# Autodesk Inventor assembly: Почти готово_CPY
(part 2 of 3)
592. Винт ГОСТ 11738-84 M 10x35:3
593. Шайба  ГОСТ 11371-78 13:6
594. Винт ГОСТ 11738-84 M 10x35:4
595. Шайба  ГОСТ 11371-78 13:7
596. Винт ГОСТ 11738-84 M 10x35:5
597. Шайба  ГОСТ 11371-78 13:8
598. Винт ГОСТ 11738-84 M 10x35:6
599. Шайба  ГОСТ 11371-78 13:9
600. Винт ГОСТ 11738-84 M 10x35:7
601. Шайба  ГОСТ 11371-78 13:10
602. Винт ГОСТ 11738-84 M 10x35:8
603. Шайба  ГОСТ 11371-78 13:11
604. Винт ГОСТ 11738-84 M 10x30:1 — Жесткий:131
605. Шайба  ГОСТ 11371-78 13:2 — Жесткий:130, Жесткий:131
606. Винт ГОСТ 11738-84 M 10x30:2
607. Шайба  ГОСТ 11371-78 13:12
608. Винт ГОСТ 11738-84 M 10x30:3
609. Шайба  ГОСТ 11371-78 13:13
610. Винт ГОСТ 11738-84 M 10x30:4
611. Шайба  ГОСТ 11371-78 13:14
612. Винт ГОСТ 11738-84 M 10x30:5
613. Шайба  ГОСТ 11371-78 13:15
614. Винт ГОСТ 11738-84 M 10x30:6
615. Шайба  ГОСТ 11371-78 13:16
616. Винт ГОСТ 11738-84 M 10x30:7
617. Шайба  ГОСТ 11371-78 13:17
618. Винт ГОСТ 11738-84 M 10x30:8
619. Шайба  ГОСТ 11371-78 13:18
620. Шайба  ГОСТ 11371-78 13:4 — Жесткий:134, Жесткий:135
621. Винт ГОСТ 11738-84 M 10x25:2 — Жесткий:135
622. Шайба  ГОСТ 11371-78 13:19
623. Винт ГОСТ 11738-84 M 10x25:3
624. Шайба  ГОСТ 11371-78 13:20
625. Винт ГОСТ 11738-84 M 10x25:4
626. Шайба  ГОСТ 11371-78 13:21
627. Винт ГОСТ 11738-84 M 10x25:5
628. Шайба  ГОСТ 11371-78 13:22
629. Винт ГОСТ 11738-84 M 10x25:6
630. Шайба  ГОСТ 11371-78 13:23
631. Винт ГОСТ 11738-84 M 10x25:7
632. Шайба  ГОСТ 11371-78 13:24
633. Винт ГОСТ 11738-84 M 10x25:8
634. Шайба  ГОСТ 11371-78 13:25
635. Винт ГОСТ 11738-84 M 10x25:9
636. Винт ГОСТ 11738-84 M 10x25:1 — Жесткий:133
637. Шайба  ГОСТ 11371-78 13:3 — Жесткий:133, Жесткий:132
638. Винт ГОСТ 11738-84 M 10x25:10
639. Шайба  ГОСТ 11371-78 13:26
640. Винт ГОСТ 11738-84 M 10x25:11
641. Шайба  ГОСТ 11371-78 13:27
642. Винт ГОСТ 11738-84 M 10x25:12
643. Шайба  ГОСТ 11371-78 13:28
644. Винт ГОСТ 11738-84 M 10x25:13
645. Шайба  ГОСТ 11371-78 13:29
646. Винт ГОСТ 11738-84 M 10x25:14
647. Шайба  ГОСТ 11371-78 13:30
648. Винт ГОСТ 11738-84 M 10x25:15
649. Шайба  ГОСТ 11371-78 13:31
650. Винт ГОСТ 11738-84 M 10x25:16
651. Шайба  ГОСТ 11371-78 13:32
652. Шпилька ГОСТ 22034-76 M20-6g×50:2 — Жесткий:122, Жесткий:124, Жесткий:123
653. Гайка ГОСТ 15521-70 M20:2 — Жесткий:124
654. Шайба ГОСТ 10450-78 19:2 — Жесткий:123
655. Шпилька ГОСТ 22034-76 M20-6g×50:14
656. Гайка ГОСТ 15521-70 M20:14
657. Шайба ГОСТ 10450-78 19:14
658. Шпилька ГОСТ 22034-76 M20-6g×50:15
659. Гайка ГОСТ 15521-70 M20:15
660. Шайба ГОСТ 10450-78 19:15
661. Шпилька ГОСТ 22034-76 M20-6g×50:16
662. Гайка ГОСТ 15521-70 M20:16
663. Шайба ГОСТ 10450-78 19:16
664. Шпилька ГОСТ 22034-76 M20-6g×50:17
665. Гайка ГОСТ 15521-70 M20:17
666. Шайба ГОСТ 10450-78 19:17
667. Шпилька ГОСТ 22034-76 M20-6g×50:18
668. Гайка ГОСТ 15521-70 M20:18
669. Шайба ГОСТ 10450-78 19:18
670. Шпилька ГОСТ 22034-76 M20-6g×50:19
671. Гайка ГОСТ 15521-70 M20:19
672. Шайба ГОСТ 10450-78 19:19
673. Шпилька ГОСТ 22034-76 M20-6g×50:20
674. Гайка ГОСТ 15521-70 M20:20
675. Шайба ГОСТ 10450-78 19:20
676. Шпилька ГОСТ 22034-76 M20-6g×50:21
677. Гайка ГОСТ 15521-70 M20:21
678. Шайба ГОСТ 10450-78 19:21
679. Шпилька ГОСТ 22034-76 M20-6g×50:22
680. Гайка ГОСТ 15521-70 M20:22
681. Шайба ГОСТ 10450-78 19:22
682. Гайка ГОСТ 15521-70 M20:3 — Жесткий:198
683. Шпилька ГОСТ 22034-76 M20-6g×50:3 — Жесткий:198, Жесткий:199
684. Шайба ГОСТ 10450-78 19:3 — Жесткий:199
685. Гайка ГОСТ 15521-70 M20:23
686. Шпилька ГОСТ 22034-76 M20-6g×50:23
687. Шайба ГОСТ 10450-78 19:23
688. Гайка ГОСТ 15521-70 M20:24
689. Шпилька ГОСТ 22034-76 M20-6g×50:24
690. Шайба ГОСТ 10450-78 19:24
691. Гайка ГОСТ 15521-70 M20:25
692. Шпилька ГОСТ 22034-76 M20-6g×50:25
693. Шайба ГОСТ 10450-78 19:25
694. Гайка ГОСТ 15521-70 M20:26
695. Шпилька ГОСТ 22034-76 M20-6g×50:26
696. Шайба ГОСТ 10450-78 19:26
697. Гайка ГОСТ 15521-70 M20:27
698. Шпилька ГОСТ 22034-76 M20-6g×50:27
699. Шайба ГОСТ 10450-78 19:27
700. Гайка ГОСТ 15521-70 M20:28
701. Шпилька ГОСТ 22034-76 M20-6g×50:28
702. Шайба ГОСТ 10450-78 19:28
703. Гайка ГОСТ 15521-70 M20:29
704. Шпилька ГОСТ 22034-76 M20-6g×50:29
705. Шайба ГОСТ 10450-78 19:29
706. Гайка ГОСТ 15521-70 M20:30
707. Шпилька ГОСТ 22034-76 M20-6g×50:30
708. Шайба ГОСТ 10450-78 19:30
709. Гайка ГОСТ 15521-70 M20:31
710. Шпилька ГОСТ 22034-76 M20-6g×50:31
711. Шайба ГОСТ 10450-78 19:31
712. Шпилька ГОСТ 22034-76 M20-6g×50:4 — Жесткий:200, Жесткий:201
713. Гайка ГОСТ 15521-70 M20:4 — Жесткий:200
714. Шайба ГОСТ 10450-78 19:4 — Жесткий:201
715. Шпилька ГОСТ 22034-76 M20-6g×50:32
716. Гайка ГОСТ 15521-70 M20:32
717. Шайба ГОСТ 10450-78 19:32
718. Шпилька ГОСТ 22034-76 M20-6g×50:33
719. Гайка ГОСТ 15521-70 M20:33
720. Шайба ГОСТ 10450-78 19:33
721. Шпилька ГОСТ 22034-76 M20-6g×50:34
722. Гайка ГОСТ 15521-70 M20:34
723. Шайба ГОСТ 10450-78 19:34
724. Шпилька ГОСТ 22034-76 M20-6g×50:35
725. Гайка ГОСТ 15521-70 M20:35
726. Шайба ГОСТ 10450-78 19:35
727. Шпилька ГОСТ 22034-76 M20-6g×50:36
728. Гайка ГОСТ 15521-70 M20:36
729. Шайба ГОСТ 10450-78 19:36
730. Шпилька ГОСТ 22034-76 M20-6g×50:37
731. Гайка ГОСТ 15521-70 M20:37
732. Шайба ГОСТ 10450-78 19:37
733. Шпилька ГОСТ 22034-76 M20-6g×50:38
734. Гайка ГОСТ 15521-70 M20:38
735. Шайба ГОСТ 10450-78 19:38
736. Шпилька ГОСТ 22034-76 M20-6g×50:39
737. Гайка ГОСТ 15521-70 M20:39
738. Шайба ГОСТ 10450-78 19:39
739. Шпилька ГОСТ 22034-76 M20-6g×50:40
740. Гайка ГОСТ 15521-70 M20:40
741. Шайба ГОСТ 10450-78 19:40
## Component patterns: (16 elements, first: Шпилька ГОСТ 22038-76 M20-6g×85:1 + Шайба ГОСТ 10450-78 21:1 + Гайка ГОСТ 15524-70 M20:1), (10 elements, first: Гайка ГОСТ 15521-70 M20:1 + Шпилька ГОСТ 22034-76 M20-6g×50:1 + Шайба ГОСТ 10450-78 19:1), (16 elements, first: Шпилька ГОСТ 22038-76 M24-6g×70:1 + Гайка ГОСТ 15524-70 M24:1 + Шайба  ГОСТ 11371-78 25:1), (8 elements, first: Винт ГОСТ 11738-84 M 10x35:1 + Шайба  ГОСТ 11371-78 13:1), (8 elements, first: Винт ГОСТ 11738-84 M 10x30:1 + Шайба  ГОСТ 11371-78 13:2), (8 elements, first: Шайба  ГОСТ 11371-78 13:4 + Винт ГОСТ 11738-84 M 10x25:2), (8 elements, first: Винт ГОСТ 11738-84 M 10x25:1 + Шайба  ГОСТ 11371-78 13:3), (10 elements, first: Шпилька ГОСТ 22034-76 M20-6g×50:2 + Гайка ГОСТ 15521-70 M20:2 + Шайба ГОСТ 10450-78 19:2), (10 elements, first: Гайка ГОСТ 15521-70 M20:3 + Шпилька ГОСТ 22034-76 M20-6g×50:3 + Шайба ГОСТ 10450-78 19:3), (10 elements, first: Шпилька ГОСТ 22034-76 M20-6g×50:4 + Гайка ГОСТ 15521-70 M20:4 + Шайба ГОСТ 10450-78 19:4)
## Relationships (407: WeldJoint 394, Flush 7, Mate 2, CylindricalJoint 2, RevoluteJoint 2)
- Совмещение:1 [Mate] (115 mm): Верхняя часть поршня_CPY:1 ↔ Крышка цилиндра 1_CPY:1
- Заподлицо:1 [Flush] (449.5 mm): Шайба  ГОСТ 11371-78 25:1
- Совмещение:2 [Mate] (449.5 mm): Шайба  ГОСТ 11371-78 25:2
- Заподлицо:2 [Flush] (-412.5 mm): Цилиндр2_CPY:1
- Заподлицо:3 [Flush] (-307 mm): Деталь6_CPY:1
- Заподлицо:5 [Flush]: Фонарь_CPY:1 ↔ Прокладка крышки фонаря 1_CPY:1
- Заподлицо:4 [Flush]: Фонарь_CPY:1 ↔ Прокладка крышки фонаря 1_CPY:1
- Заподлицо:7 [Flush]: Фонарь_CPY:1 ↔ Прокладка крышки фонаря 2_CPY:1
- Заподлицо:6 [Flush]: Фонарь_CPY:1 ↔ Прокладка крышки фонаря 2_CPY:1
- Цилиндрический:2 [CylindricalJoint]: Фонарь_CPY:1 ↔ Башмак_CPY:1
- Жесткий:4 [WeldJoint]: Башмак_CPY:1 ↔ Крейцкопф_CPY:1
- Жесткий:1 [WeldJoint]: Втулка под палец_CPY:1 ↔ Крейцкопф_CPY:1
- Жесткий:3 [WeldJoint]: Втулка палец шатун_CPY:1 ↔ Втулка под палец_CPY:2
- Жесткий:2 [WeldJoint]: Крейцкопф_CPY:1 ↔ Втулка под палец_CPY:2
- Жесткий:5 [WeldJoint]: Крейцкопф_CPY:1 ↔ Башмак_CPY:2
- С поворотом:1 [RevoluteJoint]: Втулка под палец_CPY:1 ↔ Палец_CPY:1
- Жесткий:7 [WeldJoint]: Палец_CPY:1 ↔ Стопорное кольцо_CPY:1
- Жесткий:6 [WeldJoint]: Палец_CPY:1 ↔ Стопорное кольцо_CPY:2
- Жесткий:14 [WeldJoint]: Гайка шток-поршень_CPY:1 ↔ Кольцо поршень-шток верх_CPY:1
- Жесткий:13 [WeldJoint]: Верхняя часть поршня_CPY:1 ↔ Кольцо поршень-шток верх_CPY:1
- Жесткий:9 [WeldJoint]: Верхняя часть поршня_CPY:1 ↔ Кольцо поршня_CPY:1
- С поворотом:3 [RevoluteJoint]: Корпус дросселя_CPY:1 ↔ Корпус сальника_CPY:1
- Жесткий:16 [WeldJoint]: Втулка_CPY:1 ↔ Крышка цилиндра 1_CPY:1
- Жесткий:70 [WeldJoint] (-2 mm): Фонарь_CPY:1 ↔ Крышка цилиндра 2_CPY:1
- Жесткий:12 [WeldJoint]: Кольцо поршень-шток низ_CPY:1 ↔ Нижняя часть поршня_CPY:1
- Жесткий:8 [WeldJoint]: Верхняя часть поршня_CPY:1 ↔ Нижняя часть поршня_CPY:1
- Жесткий:21 [WeldJoint]: Нижняя часть поршня_CPY:1 ↔ Опорное кольцо_CPY:1
- Жесткий:27 [WeldJoint]: Кольцо сальника_CPY:1 ↔ Пружина сальника_CPY:1
- Жесткий:79 [WeldJoint]: Крышка цилиндра 2_CPY:1 ↔ Цилиндр2_CPY:1
- Жесткий:23 [WeldJoint] (1 mm): Крышка стакана_CPY:1 ↔ Цилиндр2_CPY:1
- Жесткий:15 [WeldJoint]: Втулка_CPY:1 ↔ Цилиндр2_CPY:1
- Жесткий:11 [WeldJoint]: Нижняя часть поршня_CPY:1 ↔ Кольцо поршня_CPY:2
- Цилиндрический:1 [CylindricalJoint]: Втулка_CPY:1 ↔ Кольцо поршня_CPY:3
- Жесткий:10 [WeldJoint]: Нижняя часть поршня_CPY:1 ↔ Кольцо поршня_CPY:3
- Жесткий:80 [WeldJoint] (-2 mm): Цилиндр2_CPY:1 ↔ Клапан1_CPY:1
- Жесткий:18 [WeldJoint]: Цилиндр2_CPY:1 ↔ Прокладка клапана_CPY:1
- Жесткий:81 [WeldJoint] (-22 mm): Цилиндр2_CPY:1 ↔ Стакан1_CPY:1
- Жесткий:20 [WeldJoint]: Верхняя часть поршня_CPY:1 ↔ Опорное кольцо_CPY:2
- Жесткий:26 [WeldJoint]: Корпус дросселя_CPY:1 ↔ Дроссельное кольцо_CPY:1
- Жесткий:25 [WeldJoint] (2 mm): Пружина дросселя_CPY:1 ↔ Дроссельное кольцо_CPY:1
- Жесткий:32 [WeldJoint]: Корпус сальника_CPY:1 ↔ Кольцо сальника_CPY:2
- Жесткий:31 [WeldJoint]: Кольцо сальника_CPY:1 ↔ Кольцо сальника_CPY:2
- Жесткий:28 [WeldJoint]: Кольцо сальника_CPY:2 ↔ Пружина сальника_CPY:2
- Жесткий:30 [WeldJoint]: Кольцо сальника_CPY:1 ↔ Кольцо сальника_CPY:3
- Жесткий:29 [WeldJoint]: Кольцо сальника_CPY:3 ↔ Пружина сальника_CPY:3
- Жесткий:57 [WeldJoint]: Корпус сальника_CPY:1 ↔ Корпус сальника_CPY:2
- Жесткий:33 [WeldJoint]: Кольцо сальника_CPY:4 ↔ Пружина сальника_CPY:4
- Жесткий:38 [WeldJoint]: Корпус сальника_CPY:2 ↔ Кольцо сальника_CPY:5
- Жесткий:37 [WeldJoint]: Кольцо сальника_CPY:4 ↔ Кольцо сальника_CPY:5
- Жесткий:34 [WeldJoint]: Кольцо сальника_CPY:5 ↔ Пружина сальника_CPY:5
- Жесткий:36 [WeldJoint]: Кольцо сальника_CPY:4 ↔ Кольцо сальника_CPY:6
- Жесткий:35 [WeldJoint]: Кольцо сальника_CPY:6 ↔ Пружина сальника_CPY:6
- Жесткий:58 [WeldJoint]: Корпус сальника_CPY:2 ↔ Корпус сальника_CPY:3
- Жесткий:39 [WeldJoint]: Кольцо сальника_CPY:7 ↔ Пружина сальника_CPY:7
- Жесткий:44 [WeldJoint]: Корпус сальника_CPY:3 ↔ Кольцо сальника_CPY:8
- Жесткий:43 [WeldJoint]: Кольцо сальника_CPY:7 ↔ Кольцо сальника_CPY:8
- Жесткий:40 [WeldJoint]: Кольцо сальника_CPY:8 ↔ Пружина сальника_CPY:8
- Жесткий:42 [WeldJoint]: Кольцо сальника_CPY:7 ↔ Кольцо сальника_CPY:9
- Жесткий:41 [WeldJoint]: Кольцо сальника_CPY:9 ↔ Пружина сальника_CPY:9
- Жесткий:59 [WeldJoint]: Корпус сальника_CPY:3 ↔ Корпус сальника_CPY:4
- Жесткий:45 [WeldJoint]: Кольцо сальника_CPY:10 ↔ Пружина сальника_CPY:10
- Жесткий:50 [WeldJoint]: Корпус сальника_CPY:4 ↔ Кольцо сальника_CPY:11
- Жесткий:49 [WeldJoint]: Кольцо сальника_CPY:10 ↔ Кольцо сальника_CPY:11
- Жесткий:46 [WeldJoint]: Кольцо сальника_CPY:11 ↔ Пружина сальника_CPY:11
- Жесткий:48 [WeldJoint]: Кольцо сальника_CPY:10 ↔ Кольцо сальника_CPY:12
- Жесткий:47 [WeldJoint]: Кольцо сальника_CPY:12 ↔ Пружина сальника_CPY:12
- Жесткий:60 [WeldJoint]: Корпус сальника_CPY:4 ↔ Корпус сальника_CPY:5
- Жесткий:51 [WeldJoint]: Кольцо сальника_CPY:13 ↔ Пружина сальника_CPY:13
- Жесткий:56 [WeldJoint]: Корпус сальника_CPY:5 ↔ Кольцо сальника_CPY:14
- Жесткий:55 [WeldJoint]: Кольцо сальника_CPY:13 ↔ Кольцо сальника_CPY:14
- Жесткий:52 [WeldJoint]: Кольцо сальника_CPY:14 ↔ Пружина сальника_CPY:14
- Жесткий:54 [WeldJoint]: Кольцо сальника_CPY:13 ↔ Кольцо сальника_CPY:15
- Жесткий:53 [WeldJoint]: Кольцо сальника_CPY:15 ↔ Пружина сальника_CPY:15
- Жесткий:62 [WeldJoint] (-1 mm): Корпус дросселя_CPY:1 ↔ Уплотнительное кольцо_CPY:1
- Жесткий:61 [WeldJoint] (1 mm): Крышка цилиндра 2_CPY:1 ↔ Уплотнительное кольцо_CPY:1
- Жесткий:63 [WeldJoint]: Кольцо сальника_CPY:16 ↔ Пружина сальника_CPY:16
- Жесткий:67 [WeldJoint]: Кольцо сальника_CPY:16 ↔ Кольцо сальника_CPY:17
- Жесткий:64 [WeldJoint]: Кольцо сальника_CPY:17 ↔ Пружина сальника_CPY:17
- Жесткий:66 [WeldJoint]: Кольцо сальника_CPY:16 ↔ Кольцо сальника_CPY:18
- Жесткий:65 [WeldJoint]: Кольцо сальника_CPY:18 ↔ Пружина сальника_CPY:18
- Жесткий:69 [WeldJoint]: Фонарь_CPY:1 ↔ Уплотнение фонарь_CPY:1
- Жесткий:77 [WeldJoint]: Корпус сальника_CPY:5 ↔ Корпус сальника_CPY:6
- Жесткий:71 [WeldJoint]: Кольцо сальника_CPY:19 ↔ Пружина сальника_CPY:19
- Жесткий:76 [WeldJoint]: Корпус сальника_CPY:6 ↔ Кольцо сальника_CPY:20
- Жесткий:75 [WeldJoint]: Кольцо сальника_CPY:19 ↔ Кольцо сальника_CPY:20
- Жесткий:72 [WeldJoint]: Кольцо сальника_CPY:20 ↔ Пружина сальника_CPY:20
- Жесткий:74 [WeldJoint]: Кольцо сальника_CPY:19 ↔ Кольцо сальника_CPY:21
- Жесткий:73 [WeldJoint]: Кольцо сальника_CPY:21 ↔ Пружина сальника_CPY:21
- Жесткий:78 [WeldJoint] (3 mm): Крышка цилиндра 2_CPY:1 ↔ Крышка сальников_CPY:1
- Жесткий:95 [WeldJoint]: Корпус сальника перегородка 1_CPY:1 ↔ Крышка перегородки11_CPY:1
- Жесткий:94 [WeldJoint]: Фонарь_CPY:1 ↔ Крышка перегородки11_CPY:1
- Жесткий:96 [WeldJoint]: Корпус сальника перегородка 1_CPY:1 ↔ Крышка перегородки12_CPY:1
- Жесткий:104 [WeldJoint]: Корпус маслосъемника_CPY:1 ↔ Крышка перегородки21_CPY:1
- Жесткий:103 [WeldJoint]: Кольцо сальника_CPY:17 ↔ Крышка перегородки21_CPY:1
- Жесткий:98 [WeldJoint]: Фонарь_CPY:1 ↔ Крышка перегородки21_CPY:1
- Жесткий:105 [WeldJoint]: Крышка перегородки21_CPY:1 ↔ Крышка перегородки22_CPY:1
- Жесткий:99 [WeldJoint] (-1 mm): Маслосъемная пружина_CPY:1 ↔ Маслосъемное кольцо_CPY:1
- Жесткий:97 [WeldJoint]: Фонарь_CPY:1 ↔ Придав перегородки1_CPY:1
- Жесткий:82 [WeldJoint]: Кольцо сальника_CPY:22 ↔ Пружина сальника_CPY:22
- Жесткий:87 [WeldJoint]: Корпус сальника перегородка 1_CPY:1 ↔ Кольцо сальника_CPY:23
- Жесткий:86 [WeldJoint]: Кольцо сальника_CPY:22 ↔ Кольцо сальника_CPY:23
- Жесткий:83 [WeldJoint]: Кольцо сальника_CPY:23 ↔ Пружина сальника_CPY:23
- Жесткий:85 [WeldJoint]: Кольцо сальника_CPY:22 ↔ Кольцо сальника_CPY:24
- Жесткий:84 [WeldJoint]: Кольцо сальника_CPY:24 ↔ Пружина сальника_CPY:24
- Жесткий:88 [WeldJoint]: Кольцо сальника_CPY:25 ↔ Пружина сальника_CPY:25
- Жесткий:93 [WeldJoint]: Корпус сальника перегородка 1_CPY:1 ↔ Кольцо сальника_CPY:26
- Жесткий:92 [WeldJoint]: Кольцо сальника_CPY:25 ↔ Кольцо сальника_CPY:26
- Жесткий:89 [WeldJoint]: Кольцо сальника_CPY:26 ↔ Пружина сальника_CPY:26
- Жесткий:91 [WeldJoint]: Кольцо сальника_CPY:25 ↔ Кольцо сальника_CPY:27
- Жесткий:90 [WeldJoint]: Кольцо сальника_CPY:27 ↔ Пружина сальника_CPY:27
- Жесткий:102 [WeldJoint]: Корпус маслосъемника_CPY:1 ↔ Маслосъемное кольцо_CPY:2
- Жесткий:101 [WeldJoint]: Маслосъемное кольцо_CPY:1 ↔ Маслосъемное кольцо_CPY:2
- Жесткий:100 [WeldJoint] (-1 mm): Маслосъемная пружина_CPY:2 ↔ Маслосъемное кольцо_CPY:2
- Жесткий:106 [WeldJoint]: Фонарь_CPY:1 ↔ Придав перегородки1_CPY:2
- Жесткий:110 [WeldJoint] (-3.5 mm): Гайка шток_CPY:1 ↔ Шток_CPY:1
- Жесткий:107 [WeldJoint] (4.75 mm): Гайка шток-поршень_CPY:1 ↔ Шток_CPY:1
- Жесткий:207 [WeldJoint]: Фланецгайка_CPY:1 ↔ Прокладка крейцкопф_CPY:1
- Жесткий:206 [WeldJoint]: Крейцкопф_CPY:1 ↔ Прокладка крейцкопф_CPY:1
- Жесткий:112 [WeldJoint]: Крышка цилиндра 1_CPY:1 ↔ Шайба  ГОСТ 11371-78 25:1
- Жесткий:113 [WeldJoint] (-8.75 mm): Шпилька ГОСТ 22038-76 M24-6g×70:1 ↔ Гайка ГОСТ 15524-70 M24:1
- Жесткий:111 [WeldJoint]: Цилиндр2_CPY:1 ↔ Шпилька ГОСТ 22038-76 M24-6g×70:1
- Жесткий:114 [WeldJoint] (-8.75 mm): Шпилька ГОСТ 22038-76 M24-6g×70:2 ↔ Гайка ГОСТ 15524-70 M24:2
- Жесткий:116 [WeldJoint] (-2 mm): Цилиндр2_CPY:1 ↔ Клапан1_CPY:2
- Жесткий:115 [WeldJoint]: Цилиндр2_CPY:1 ↔ Прокладка клапана_CPY:2
- Жесткий:117 [WeldJoint] (-22 mm): Цилиндр2_CPY:1 ↔ Стакан1_CPY:2
- Жесткий:118 [WeldJoint] (1 mm): Цилиндр2_CPY:1 ↔ Крышка стакана_CPY:2
- Жесткий:119 [WeldJoint] (-1 mm): Цилиндр2_CPY:1 ↔ Шпилька ГОСТ 22034-76 M20-6g×50:1
- Жесткий:121 [WeldJoint] (-2.5 mm): Гайка ГОСТ 15521-70 M20:1 ↔ Шпилька ГОСТ 22034-76 M20-6g×50:1
- Жесткий:120 [WeldJoint] (-20 mm): Шпилька ГОСТ 22034-76 M20-6g×50:1 ↔ Шайба ГОСТ 10450-78 19:1
- Жесткий:122 [WeldJoint]: Цилиндр2_CPY:1 ↔ Шпилька ГОСТ 22034-76 M20-6g×50:2
- Жесткий:124 [WeldJoint] (-2.25 mm): Шпилька ГОСТ 22034-76 M20-6g×50:2 ↔ Гайка ГОСТ 15521-70 M20:2
- Жесткий:123 [WeldJoint] (-20 mm): Шпилька ГОСТ 22034-76 M20-6g×50:2 ↔ Шайба ГОСТ 10450-78 19:2
- Жесткий:127 [WeldJoint] (-2 mm): Фонарь_CPY:1 ↔ Гайка ГОСТ 15524-70 M20:1
- Жесткий:126 [WeldJoint] (-32 mm): Шпилька ГОСТ 22038-76 M20-6g×85:1 ↔ Шайба ГОСТ 10450-78 21:1
- Жесткий:125 [WeldJoint]: Крышка цилиндра 2_CPY:1 ↔ Шпилька ГОСТ 22038-76 M20-6g×85:1
- Жесткий:130 [WeldJoint]: Крышка перегородки22_CPY:1 ↔ Шайба  ГОСТ 11371-78 13:2
- Жесткий:134 [WeldJoint]: Придав перегородки1_CPY:1 ↔ Шайба  ГОСТ 11371-78 13:4
- Жесткий:128 [WeldJoint]: Крышка перегородки12_CPY:1 ↔ Шайба  ГОСТ 11371-78 13:1
- Жесткий:135 [WeldJoint]: Шайба  ГОСТ 11371-78 13:4 ↔ Винт ГОСТ 11738-84 M 10x25:2
- Жесткий:133 [WeldJoint]: Винт ГОСТ 11738-84 M 10x25:1 ↔ Шайба  ГОСТ 11371-78 13:3
- Жесткий:132 [WeldJoint]: Придав перегородки1_CPY:2 ↔ Шайба  ГОСТ 11371-78 13:3
- Жесткий:129 [WeldJoint]: Винт ГОСТ 11738-84 M 10x35:1 ↔ Шайба  ГОСТ 11371-78 13:1
- Жесткий:131 [WeldJoint]: Винт ГОСТ 11738-84 M 10x30:1 ↔ Шайба  ГОСТ 11371-78 13:2
- Жесткий:138 [WeldJoint] (-38 mm): Шпилька ГОСТ 22038-76 M24-6g×80:1 ↔ Гайка ГОСТ 15524-70 M24:18
- Жесткий:137 [WeldJoint] (-38 mm): Шпилька ГОСТ 22038-76 M24-6g×80:1 ↔ Шайба  ГОСТ 11371-78 28:1
- Жесткий:140 [WeldJoint] (-38 mm): Шпилька ГОСТ 22038-76 M24-6g×80:2 ↔ Гайка ГОСТ 15524-70 M24:19
- Жесткий:163 [WeldJoint]: Фонарь_CPY:1 ↔ Шайба  ГОСТ 11371-78 28:2
- Жесткий:139 [WeldJoint] (-38 mm): Шпилька ГОСТ 22038-76 M24-6g×80:2 ↔ Шайба  ГОСТ 11371-78 28:2
- Жесткий:142 [WeldJoint] (-38 mm): Шпилька ГОСТ 22038-76 M24-6g×80:3 ↔ Гайка ГОСТ 15524-70 M24:20
- Жесткий:165 [WeldJoint]: Фонарь_CPY:1 ↔ Шайба  ГОСТ 11371-78 28:3
- Жесткий:141 [WeldJoint] (-38 mm): Шпилька ГОСТ 22038-76 M24-6g×80:3 ↔ Шайба  ГОСТ 11371-78 28:3
- Жесткий:144 [WeldJoint] (-38 mm): Шпилька ГОСТ 22038-76 M24-6g×80:4 ↔ Гайка ГОСТ 15524-70 M24:21
- Жесткий:166 [WeldJoint]: Фонарь_CPY:1 ↔ Шайба  ГОСТ 11371-78 28:4
- Жесткий:143 [WeldJoint] (-38 mm): Шпилька ГОСТ 22038-76 M24-6g×80:4 ↔ Шайба  ГОСТ 11371-78 28:4
- Жесткий:146 [WeldJoint] (-38 mm): Шпилька ГОСТ 22038-76 M24-6g×80:5 ↔ Гайка ГОСТ 15524-70 M24:22
- Жесткий:164 [WeldJoint]: Фонарь_CPY:1 ↔ Шайба  ГОСТ 11371-78 28:5
- Жесткий:145 [WeldJoint] (-38 mm): Шпилька ГОСТ 22038-76 M24-6g×80:5 ↔ Шайба  ГОСТ 11371-78 28:5
- Жесткий:148 [WeldJoint] (-38 mm): Шпилька ГОСТ 22038-76 M24-6g×80:6 ↔ Гайка ГОСТ 15524-70 M24:23
- Жесткий:171 [WeldJoint]: Фонарь_CPY:1 ↔ Шайба  ГОСТ 11371-78 28:6
- Жесткий:147 [WeldJoint] (-38 mm): Шпилька ГОСТ 22038-76 M24-6g×80:6 ↔ Шайба  ГОСТ 11371-78 28:6
- Жесткий:150 [WeldJoint] (-38 mm): Шпилька ГОСТ 22038-76 M24-6g×80:7 ↔ Гайка ГОСТ 15524-70 M24:24
- Жесткий:173 [WeldJoint]: Фонарь_CPY:1 ↔ Шайба  ГОСТ 11371-78 28:7
- Жесткий:149 [WeldJoint] (-38 mm): Шпилька ГОСТ 22038-76 M24-6g×80:7 ↔ Шайба  ГОСТ 11371-78 28:7
- Жесткий:152 [WeldJoint] (-38 mm): Шпилька ГОСТ 22038-76 M24-6g×80:8 ↔ Гайка ГОСТ 15524-70 M24:25
- Жесткий:174 [WeldJoint]: Фонарь_CPY:1 ↔ Шайба  ГОСТ 11371-78 28:8
- Жесткий:151 [WeldJoint] (-38 mm): Шпилька ГОСТ 22038-76 M24-6g×80:8 ↔ Шайба  ГОСТ 11371-78 28:8
- Жесткий:154 [WeldJoint] (-38 mm): Шпилька ГОСТ 22038-76 M24-6g×80:9 ↔ Гайка ГОСТ 15524-70 M24:26
- Жесткий:172 [WeldJoint]: Фонарь_CPY:1 ↔ Шайба  ГОСТ 11371-78 28:9
- Жесткий:153 [WeldJoint] (-38 mm): Шпилька ГОСТ 22038-76 M24-6g×80:9 ↔ Шайба  ГОСТ 11371-78 28:9
- Жесткий:156 [WeldJoint] (-38 mm): Шпилька ГОСТ 22038-76 M24-6g×80:10 ↔ Гайка ГОСТ 15524-70 M24:27
- Жесткий:169 [WeldJoint]: Фонарь_CPY:1 ↔ Шайба  ГОСТ 11371-78 28:10
- Жесткий:155 [WeldJoint] (-38 mm): Шпилька ГОСТ 22038-76 M24-6g×80:10 ↔ Шайба  ГОСТ 11371-78 28:10
- Жесткий:158 [WeldJoint] (-38 mm): Шпилька ГОСТ 22038-76 M24-6g×80:11 ↔ Гайка ГОСТ 15524-70 M24:28
- Жесткий:167 [WeldJoint]: Фонарь_CPY:1 ↔ Шайба  ГОСТ 11371-78 28:11
- Жесткий:157 [WeldJoint] (-38 mm): Шпилька ГОСТ 22038-76 M24-6g×80:11 ↔ Шайба  ГОСТ 11371-78 28:11
- Жесткий:160 [WeldJoint] (-38 mm): Шпилька ГОСТ 22038-76 M24-6g×80:12 ↔ Гайка ГОСТ 15524-70 M24:29
- Жесткий:170 [WeldJoint]: Фонарь_CPY:1 ↔ Шайба  ГОСТ 11371-78 28:12
- Жесткий:159 [WeldJoint] (-38 mm): Шпилька ГОСТ 22038-76 M24-6g×80:12 ↔ Шайба  ГОСТ 11371-78 28:12
- Жесткий:162 [WeldJoint] (-38 mm): Шпилька ГОСТ 22038-76 M24-6g×80:13 ↔ Гайка ГОСТ 15524-70 M24:30
- Жесткий:168 [WeldJoint]: Фонарь_CPY:1 ↔ Шайба  ГОСТ 11371-78 28:13
- Жесткий:161 [WeldJoint] (-38 mm): Шпилька ГОСТ 22038-76 M24-6g×80:13 ↔ Шайба  ГОСТ 11371-78 28:13
- Жесткий:176 [WeldJoint] (-38 mm): Шпилька ГОСТ 22038-76 M24-6g×80:14 ↔ Гайка ГОСТ 15524-70 M24:31
- Жесткий:192 [WeldJoint]: Фонарь_CPY:1 ↔ Шайба  ГОСТ 11371-78 28:14
- Жесткий:175 [WeldJoint] (-38 mm): Шпилька ГОСТ 22038-76 M24-6g×80:14 ↔ Шайба  ГОСТ 11371-78 28:14
- Жесткий:178 [WeldJoint] (-38 mm): Шпилька ГОСТ 22038-76 M24-6g×80:15 ↔ Гайка ГОСТ 15524-70 M24:32
- Жесткий:197 [WeldJoint]: Фонарь_CPY:1 ↔ Шайба  ГОСТ 11371-78 28:15
- Жесткий:177 [WeldJoint] (-38 mm): Шпилька ГОСТ 22038-76 M24-6g×80:15 ↔ Шайба  ГОСТ 11371-78 28:15
- Жесткий:180 [WeldJoint] (-38 mm): Шпилька ГОСТ 22038-76 M24-6g×80:16 ↔ Гайка ГОСТ 15524-70 M24:33
- Жесткий:191 [WeldJoint]: Фонарь_CPY:1 ↔ Шайба  ГОСТ 11371-78 28:16
- Жесткий:179 [WeldJoint] (-38 mm): Шпилька ГОСТ 22038-76 M24-6g×80:16 ↔ Шайба  ГОСТ 11371-78 28:16
- Жесткий:184 [WeldJoint] (-38 mm): Шпилька ГОСТ 22038-76 M24-6g×80:17 ↔ Гайка ГОСТ 15524-70 M24:34
- Жесткий:196 [WeldJoint]: Фонарь_CPY:1 ↔ Шайба  ГОСТ 11371-78 28:17
- Жесткий:183 [WeldJoint] (-38 mm): Шпилька ГОСТ 22038-76 M24-6g×80:17 ↔ Шайба  ГОСТ 11371-78 28:17
- Жесткий:186 [WeldJoint] (-38 mm): Шпилька ГОСТ 22038-76 M24-6g×80:18 ↔ Гайка ГОСТ 15524-70 M24:35
- Жесткий:194 [WeldJoint]: Фонарь_CPY:1 ↔ Шайба  ГОСТ 11371-78 28:18
- Жесткий:185 [WeldJoint] (-38 mm): Шпилька ГОСТ 22038-76 M24-6g×80:18 ↔ Шайба  ГОСТ 11371-78 28:18
- Жесткий:188 [WeldJoint] (-38 mm): Шпилька ГОСТ 22038-76 M24-6g×80:19 ↔ Гайка ГОСТ 15524-70 M24:36
- Жесткий:193 [WeldJoint]: Фонарь_CPY:1 ↔ Шайба  ГОСТ 11371-78 28:19
- Жесткий:187 [WeldJoint] (-38 mm): Шпилька ГОСТ 22038-76 M24-6g×80:19 ↔ Шайба  ГОСТ 11371-78 28:19
- Жесткий:190 [WeldJoint] (-38 mm): Шпилька ГОСТ 22038-76 M24-6g×80:20 ↔ Гайка ГОСТ 15524-70 M24:37
- Жесткий:195 [WeldJoint]: Фонарь_CPY:1 ↔ Шайба  ГОСТ 11371-78 28:20
- Жесткий:189 [WeldJoint] (-38 mm): Шпилька ГОСТ 22038-76 M24-6g×80:20 ↔ Шайба  ГОСТ 11371-78 28:20
- Жесткий:198 [WeldJoint] (-2.5 mm): Гайка ГОСТ 15521-70 M20:3 ↔ Шпилька ГОСТ 22034-76 M20-6g×50:3
- Жесткий:199 [WeldJoint] (-20 mm): Шпилька ГОСТ 22034-76 M20-6g×50:3 ↔ Шайба ГОСТ 10450-78 19:3
- Жесткий:200 [WeldJoint] (-2.25 mm): Шпилька ГОСТ 22034-76 M20-6g×50:4 ↔ Гайка ГОСТ 15521-70 M20:4
- Жесткий:201 [WeldJoint] (-20 mm): Шпилька ГОСТ 22034-76 M20-6g×50:4 ↔ Шайба ГОСТ 10450-78 19:4
- Жесткий:202 [WeldJoint]: Цилиндр2_CPY:1 ↔ Деталь5_CPY:1
- Жесткий:203 [WeldJoint]: Деталь5_CPY:1 ↔ Деталь6_CPY:1
- Жесткий:204 [WeldJoint]: Цилиндр2_CPY:1 ↔ Деталь5_CPY:2
- Жесткий:205 [WeldJoint]: Деталь5_CPY:2 ↔ Деталь6_CPY:2
- Жесткий:208 [WeldJoint]: Крейцкопф_CPY:1 ↔ Шпилька ГОСТ 22038-76 M20-6g×85:2
- Жесткий:209 [WeldJoint]: Крейцкопф_CPY:1 ↔ Шпилька ГОСТ 22038-76 M20-6g×85:3
- Жесткий:211 [WeldJoint] (-26 mm): Шпилька ГОСТ 22038-76 M20-6g×85:2 ↔ Гайка ГОСТ 15524-70 M20:2
- Жесткий:210 [WeldJoint] (-26 mm): Шпилька ГОСТ 22038-76 M20-6g×85:2 ↔ Шайба  ГОСТ 11371-78 23:1
- Жесткий:213 [WeldJoint] (-2 mm): Шпилька ГОСТ 22038-76 M20-6g×85:3 ↔ Гайка ГОСТ 15524-70 M20:3
- Жесткий:212 [WeldJoint] (-26 mm): Шпилька ГОСТ 22038-76 M20-6g×85:3 ↔ Шайба  ГОСТ 11371-78 23:2
- Жесткий:239 [WeldJoint]: Деталь6_CPY:1 ↔ Болт ГОСТ Р 50274-92 M8-6g×16-F:1
- Жесткий:233 [WeldJoint]: Деталь6_CPY:1 ↔ Болт ГОСТ Р 50274-92 M8-6g×16-F:2
- Жесткий:232 [WeldJoint]: Деталь6_CPY:1 ↔ Болт ГОСТ Р 50274-92 M8-6g×16-F:3
- Жесткий:214 [WeldJoint]: Деталь6_CPY:1 ↔ Болт ГОСТ Р 50274-92 M8-6g×16-F:4
- Жесткий:215 [WeldJoint]: Деталь6_CPY:1 ↔ Болт ГОСТ Р 50274-92 M8-6g×16-F:5
- Жесткий:223 [WeldJoint]: Деталь6_CPY:1 ↔ Болт ГОСТ Р 50274-92 M8-6g×16-F:6
- Жесткий:222 [WeldJoint]: Деталь6_CPY:1 ↔ Болт ГОСТ Р 50274-92 M8-6g×16-F:7
- Жесткий:240 [WeldJoint]: Деталь6_CPY:1 ↔ Болт ГОСТ Р 50274-92 M8-6g×16-F:8
- Жесткий:238 [WeldJoint]: Деталь6_CPY:1 ↔ Болт ГОСТ Р 50274-92 M8-6g×16-F:9
- Жесткий:236 [WeldJoint]: Деталь6_CPY:1 ↔ Болт ГОСТ Р 50274-92 M8-6g×16-F:10
- Жесткий:218 [WeldJoint]: Деталь6_CPY:1 ↔ Болт ГОСТ Р 50274-92 M8-6g×16-F:11
- Жесткий:217 [WeldJoint]: Деталь6_CPY:1 ↔ Болт ГОСТ Р 50274-92 M8-6g×16-F:12
- Жесткий:216 [WeldJoint]: Деталь6_CPY:1 ↔ Болт ГОСТ Р 50274-92 M8-6g×16-F:13
- Жесткий:237 [WeldJoint]: Деталь6_CPY:1 ↔ Болт ГОСТ Р 50274-92 M8-6g×16-F:14
- Жесткий:235 [WeldJoint]: Деталь6_CPY:1 ↔ Болт ГОСТ Р 50274-92 M8-6g×16-F:15
- Жесткий:234 [WeldJoint]: Деталь6_CPY:1 ↔ Болт ГОСТ Р 50274-92 M8-6g×16-F:16
- Жесткий:227 [WeldJoint]: Деталь6_CPY:1 ↔ Болт ГОСТ Р 50274-92 M8-6g×16-F:17
- Жесткий:226 [WeldJoint]: Деталь6_CPY:1 ↔ Болт ГОСТ Р 50274-92 M8-6g×16-F:18
- Жесткий:225 [WeldJoint]: Деталь6_CPY:1 ↔ Болт ГОСТ Р 50274-92 M8-6g×16-F:19
- Жесткий:241 [WeldJoint]: Деталь6_CPY:1 ↔ Болт ГОСТ Р 50274-92 M8-6g×16-F:20
- Жесткий:244 [WeldJoint]: Деталь6_CPY:1 ↔ Болт ГОСТ Р 50274-92 M8-6g×16-F:21
- Жесткий:231 [WeldJoint]: Деталь6_CPY:1 ↔ Болт ГОСТ Р 50274-92 M8-6g×16-F:22
- Жесткий:229 [WeldJoint]: Деталь6_CPY:1 ↔ Болт ГОСТ Р 50274-92 M8-6g×16-F:23
- Жесткий:228 [WeldJoint]: Деталь6_CPY:1 ↔ Болт ГОСТ Р 50274-92 M8-6g×16-F:24
- Жесткий:224 [WeldJoint]: Деталь6_CPY:1 ↔ Болт ГОСТ Р 50274-92 M8-6g×16-F:25
- Жесткий:243 [WeldJoint]: Деталь6_CPY:1 ↔ Болт ГОСТ Р 50274-92 M8-6g×16-F:26
- Жесткий:242 [WeldJoint]: Деталь6_CPY:1 ↔ Болт ГОСТ Р 50274-92 M8-6g×16-F:27
- Жесткий:219 [WeldJoint]: Деталь6_CPY:1 ↔ Болт ГОСТ Р 50274-92 M8-6g×16-F:28
- Жесткий:221 [WeldJoint]: Деталь6_CPY:1 ↔ Болт ГОСТ Р 50274-92 M8-6g×16-F:29
- Жесткий:220 [WeldJoint]: Деталь6_CPY:1 ↔ Болт ГОСТ Р 50274-92 M8-6g×16-F:30
- Жесткий:245 [WeldJoint]: Деталь6_CPY:1 ↔ Болт ГОСТ Р 50274-92 M8-6g×16-F:31
- Жесткий:230 [WeldJoint]: Деталь6_CPY:1 ↔ Болт ГОСТ Р 50274-92 M8-6g×16-F:32
- Жесткий:246 [WeldJoint]: Крышка фонаря 1_CPY:1 ↔ Прокладка крышки фонаря 1_CPY:1
- Жесткий:247 [WeldJoint]: Крышка фонаря 2_CPY:1 ↔ Прокладка крышки фонаря 2_CPY:1
- Жесткий:249 [WeldJoint]: Крышка фонаря 1_CPY:1 ↔ Болт ГОСТ Р 50274-92 M8-6g×16-F:65
- Жесткий:248 [WeldJoint]: Крышка фонаря 1_CPY:1 ↔ Болт ГОСТ Р 50274-92 M8-6g×16-F:66
- Жесткий:250 [WeldJoint]: Крышка фонаря 1_CPY:1 ↔ Болт ГОСТ Р 50274-92 M8-6g×16-F:67
- Жесткий:251 [WeldJoint]: Крышка фонаря 1_CPY:1 ↔ Болт ГОСТ Р 50274-92 M8-6g×16-F:68
- Жесткий:254 [WeldJoint]: Крышка фонаря 1_CPY:1 ↔ Болт ГОСТ Р 50274-92 M8-6g×16-F:69
- Жесткий:252 [WeldJoint]: Крышка фонаря 1_CPY:1 ↔ Болт ГОСТ Р 50274-92 M8-6g×16-F:70
- Жесткий:258 [WeldJoint]: Крышка фонаря 1_CPY:1 ↔ Болт ГОСТ Р 50274-92 M8-6g×16-F:71
- Жесткий:256 [WeldJoint]: Крышка фонаря 1_CPY:1 ↔ Болт ГОСТ Р 50274-92 M8-6g×16-F:72
- Жесткий:255 [WeldJoint]: Крышка фонаря 1_CPY:1 ↔ Болт ГОСТ Р 50274-92 M8-6g×16-F:73
- Жесткий:253 [WeldJoint]: Крышка фонаря 1_CPY:1 ↔ Болт ГОСТ Р 50274-92 M8-6g×16-F:74
- Жесткий:267 [WeldJoint]: Крышка фонаря 1_CPY:1 ↔ Болт ГОСТ Р 50274-92 M8-6g×16-F:75
- Жесткий:266 [WeldJoint]: Крышка фонаря 1_CPY:1 ↔ Болт ГОСТ Р 50274-92 M8-6g×16-F:76
- Жесткий:269 [WeldJoint]: Крышка фонаря 1_CPY:1 ↔ Болт ГОСТ Р 50274-92 M8-6g×16-F:77
- Жесткий:265 [WeldJoint]: Крышка фонаря 1_CPY:1 ↔ Болт ГОСТ Р 50274-92 M8-6g×16-F:78
- Жесткий:273 [WeldJoint]: Крышка фонаря 1_CPY:1 ↔ Болт ГОСТ Р 50274-92 M8-6g×16-F:79
- Жесткий:271 [WeldJoint]: Крышка фонаря 1_CPY:1 ↔ Болт ГОСТ Р 50274-92 M8-6g×16-F:80
- Жесткий:270 [WeldJoint]: Крышка фонаря 1_CPY:1 ↔ Болт ГОСТ Р 50274-92 M8-6g×16-F:81
- Жесткий:268 [WeldJoint]: Крышка фонаря 1_CPY:1 ↔ Болт ГОСТ Р 50274-92 M8-6g×16-F:82
- Жесткий:257 [WeldJoint]: Крышка фонаря 1_CPY:1 ↔ Болт ГОСТ Р 50274-92 M8-6g×16-F:83
- Жесткий:259 [WeldJoint]: Крышка фонаря 1_CPY:1 ↔ Болт ГОСТ Р 50274-92 M8-6g×16-F:84
- Жесткий:261 [WeldJoint]: Крышка фонаря 1_CPY:1 ↔ Болт ГОСТ Р 50274-92 M8-6g×16-F:85
- Жесткий:264 [WeldJoint]: Крышка фонаря 1_CPY:1 ↔ Болт ГОСТ Р 50274-92 M8-6g×16-F:86
- Жесткий:263 [WeldJoint]: Крышка фонаря 1_CPY:1 ↔ Болт ГОСТ Р 50274-92 M8-6g×16-F:87
- Жесткий:262 [WeldJoint]: Крышка фонаря 1_CPY:1 ↔ Болт ГОСТ Р 50274-92 M8-6g×16-F:88
- Жесткий:260 [WeldJoint]: Крышка фонаря 1_CPY:1 ↔ Болт ГОСТ Р 50274-92 M8-6g×16-F:89
- Жесткий:280 [WeldJoint]: Крышка фонаря 2_CPY:1 ↔ Болт ГОСТ Р 50274-92 M8-6g×16-F:90
- Жесткий:281 [WeldJoint]: Крышка фонаря 2_CPY:1 ↔ Болт ГОСТ Р 50274-92 M8-6g×16-F:91
- Жесткий:279 [WeldJoint]: Крышка фонаря 2_CPY:1 ↔ Болт ГОСТ Р 50274-92 M8-6g×16-F:92
- Жесткий:276 [WeldJoint]: Крышка фонаря 2_CPY:1 ↔ Болт ГОСТ Р 50274-92 M8-6g×16-F:93
- Жесткий:295 [WeldJoint]: Крышка фонаря 2_CPY:1 ↔ Болт ГОСТ Р 50274-92 M8-6g×16-F:94
- Жесткий:296 [WeldJoint]: Крышка фонаря 2_CPY:1 ↔ Болт ГОСТ Р 50274-92 M8-6g×16-F:95
- Жесткий:282 [WeldJoint]: Крышка фонаря 2_CPY:1 ↔ Болт ГОСТ Р 50274-92 M8-6g×16-F:96
- Жесткий:278 [WeldJoint]: Крышка фонаря 2_CPY:1 ↔ Болт ГОСТ Р 50274-92 M8-6g×16-F:97
- Жесткий:277 [WeldJoint]: Крышка фонаря 2_CPY:1 ↔ Болт ГОСТ Р 50274-92 M8-6g×16-F:98
- Жесткий:308 [WeldJoint]: Крышка фонаря 2_CPY:1 ↔ Болт ГОСТ Р 50274-92 M8-6g×16-F:99
- Жесткий:274 [WeldJoint]: Крышка фонаря 1_CPY:1 ↔ Болт ГОСТ Р 50274-92 M8-6g×16-F:100
- Жесткий:272 [WeldJoint]: Крышка фонаря 1_CPY:1 ↔ Болт ГОСТ Р 50274-92 M8-6g×16-F:101
- Жесткий:317 [WeldJoint]: Крышка фонаря 2_CPY:1 ↔ Болт ГОСТ Р 50274-92 M8-6g×16-F:102
- Жесткий:318 [WeldJoint]: Крышка фонаря 2_CPY:1 ↔ Болт ГОСТ Р 50274-92 M8-6g×16-F:103
- Жесткий:316 [WeldJoint]: Крышка фонаря 2_CPY:1 ↔ Болт ГОСТ Р 50274-92 M8-6g×16-F:104
- Жесткий:275 [WeldJoint]: Крышка фонаря 1_CPY:1 ↔ Болт ГОСТ Р 50274-92 M8-6g×16-F:105
- Жесткий:310 [WeldJoint]: Крышка фонаря 2_CPY:1 ↔ Болт ГОСТ Р 50274-92 M8-6g×16-F:106
- Жесткий:294 [WeldJoint]: Крышка фонаря 2_CPY:1 ↔ Болт ГОСТ Р 50274-92 M8-6g×16-F:107
- Жесткий:311 [WeldJoint]: Крышка фонаря 2_CPY:1 ↔ Болт ГОСТ Р 50274-92 M8-6g×16-F:108
- Жесткий:307 [WeldJoint]: Крышка фонаря 2_CPY:1 ↔ Болт ГОСТ Р 50274-92 M8-6g×16-F:109
- Жесткий:313 [WeldJoint]: Крышка фонаря 2_CPY:1 ↔ Болт ГОСТ Р 50274-92 M8-6g×16-F:110
- Жесткий:314 [WeldJoint]: Крышка фонаря 2_CPY:1 ↔ Болт ГОСТ Р 50274-92 M8-6g×16-F:111
- Жесткий:315 [WeldJoint]: Крышка фонаря 2_CPY:1 ↔ Болт ГОСТ Р 50274-92 M8-6g×16-F:112
- Жесткий:293 [WeldJoint]: Крышка фонаря 2_CPY:1 ↔ Болт ГОСТ Р 50274-92 M8-6g×16-F:113
- Жесткий:320 [WeldJoint]: Крышка фонаря 2_CPY:1 ↔ Болт ГОСТ Р 50274-92 M8-6g×16-F:114
- Жесткий:300 [WeldJoint]: Крышка фонаря 2_CPY:1 ↔ Болт ГОСТ Р 50274-92 M8-6g×16-F:115
- Жесткий:299 [WeldJoint]: Крышка фонаря 2_CPY:1 ↔ Болт ГОСТ Р 50274-92 M8-6g×16-F:116
- Жесткий:285 [WeldJoint]: Крышка фонаря 2_CPY:1 ↔ Болт ГОСТ Р 50274-92 M8-6g×16-F:117
- Жесткий:301 [WeldJoint]: Крышка фонаря 2_CPY:1 ↔ Болт ГОСТ Р 50274-92 M8-6g×16-F:118
- Жесткий:291 [WeldJoint]: Крышка фонаря 2_CPY:1 ↔ Болт ГОСТ Р 50274-92 M8-6g×16-F:119
- Жесткий:284 [WeldJoint]: Крышка фонаря 2_CPY:1 ↔ Болт ГОСТ Р 50274-92 M8-6g×16-F:120
- Жесткий:309 [WeldJoint]: Крышка фонаря 2_CPY:1 ↔ Болт ГОСТ Р 50274-92 M8-6g×16-F:121
- Жесткий:289 [WeldJoint]: Крышка фонаря 2_CPY:1 ↔ Болт ГОСТ Р 50274-92 M8-6g×16-F:122
- Жесткий:306 [WeldJoint]: Крышка фонаря 2_CPY:1 ↔ Болт ГОСТ Р 50274-92 M8-6g×16-F:123
- Жесткий:297 [WeldJoint]: Крышка фонаря 2_CPY:1 ↔ Болт ГОСТ Р 50274-92 M8-6g×16-F:124
- Жесткий:312 [WeldJoint]: Крышка фонаря 2_CPY:1 ↔ Болт ГОСТ Р 50274-92 M8-6g×16-F:125
- Жесткий:288 [WeldJoint]: Крышка фонаря 2_CPY:1 ↔ Болт ГОСТ Р 50274-92 M8-6g×16-F:126
- Жесткий:319 [WeldJoint]: Крышка фонаря 2_CPY:1 ↔ Болт ГОСТ Р 50274-92 M8-6g×16-F:127
- Жесткий:303 [WeldJoint]: Крышка фонаря 2_CPY:1 ↔ Болт ГОСТ Р 50274-92 M8-6g×16-F:128
- Жесткий:292 [WeldJoint]: Крышка фонаря 2_CPY:1 ↔ Болт ГОСТ Р 50274-92 M8-6g×16-F:129
- Жесткий:304 [WeldJoint]: Крышка фонаря 2_CPY:1 ↔ Болт ГОСТ Р 50274-92 M8-6g×16-F:130
- Жесткий:305 [WeldJoint]: Крышка фонаря 2_CPY:1 ↔ Болт ГОСТ Р 50274-92 M8-6g×16-F:131
- Жесткий:298 [WeldJoint]: Крышка фонаря 2_CPY:1 ↔ Болт ГОСТ Р 50274-92 M8-6g×16-F:132
- Жесткий:302 [WeldJoint]: Крышка фонаря 2_CPY:1 ↔ Болт ГОСТ Р 50274-92 M8-6g×16-F:133
- Жесткий:283 [WeldJoint]: Крышка фонаря 2_CPY:1 ↔ Болт ГОСТ Р 50274-92 M8-6g×16-F:134
- Жесткий:290 [WeldJoint]: Крышка фонаря 2_CPY:1 ↔ Болт ГОСТ Р 50274-92 M8-6g×16-F:135
- Жесткий:286 [WeldJoint]: Крышка фонаря 2_CPY:1 ↔ Болт ГОСТ Р 50274-92 M8-6g×16-F:136
- Жесткий:287 [WeldJoint]: Крышка фонаря 2_CPY:1 ↔ Болт ГОСТ Р 50274-92 M8-6g×16-F:137
- Жесткий:321 [WeldJoint]: Крышка фонаря 2_CPY:1 ↔ Болт ГОСТ Р 50274-92 M8-6g×16-F:138
- Жесткий:323 [WeldJoint]: Крышка фонаря 2_CPY:1 ↔ Болт ГОСТ Р 50274-92 M8-6g×16-F:139
- Жесткий:322 [WeldJoint]: Крышка фонаря 2_CPY:1 ↔ Болт ГОСТ Р 50274-92 M8-6g×16-F:140
- Жесткий:324 [WeldJoint]: Крышка фонаря 2_CPY:1 ↔ Болт ГОСТ Р 50274-92 M8-6g×16-F:141
- Жесткий:325 [WeldJoint]: Крышка фонаря 1_MIR_CPY:1 ↔ Прокладка крышки фонаря 1_MIR_CPY:1
- Жесткий:326 [WeldJoint]: Крышка фонаря 2_MIR_CPY:1 ↔ Прокладка крышки фонаря 2_MIR_CPY:1
- Жесткий:327 [WeldJoint]: Крышка фонаря 1_MIR_CPY:1 ↔ Болт ГОСТ Р 50274-92 M8-6g×16-F:142
- Жесткий:328 [WeldJoint]: Крышка фонаря 1_MIR_CPY:1 ↔ Болт ГОСТ Р 50274-92 M8-6g×16-F:143
- Жесткий:329 [WeldJoint]: Крышка фонаря 1_MIR_CPY:1 ↔ Болт ГОСТ Р 50274-92 M8-6g×16-F:144
- Жесткий:330 [WeldJoint]: Крышка фонаря 1_MIR_CPY:1 ↔ Болт ГОСТ Р 50274-92 M8-6g×16-F:145
- Жесткий:331 [WeldJoint]: Крышка фонаря 1_MIR_CPY:1 ↔ Болт ГОСТ Р 50274-92 M8-6g×16-F:146
- Жесткий:332 [WeldJoint]: Крышка фонаря 1_MIR_CPY:1 ↔ Болт ГОСТ Р 50274-92 M8-6g×16-F:147
- Жесткий:333 [WeldJoint]: Крышка фонаря 1_MIR_CPY:1 ↔ Болт ГОСТ Р 50274-92 M8-6g×16-F:148
- Жесткий:334 [WeldJoint]: Крышка фонаря 1_MIR_CPY:1 ↔ Болт ГОСТ Р 50274-92 M8-6g×16-F:149
- Жесткий:335 [WeldJoint]: Крышка фонаря 1_MIR_CPY:1 ↔ Болт ГОСТ Р 50274-92 M8-6g×16-F:150
- Жесткий:336 [WeldJoint]: Крышка фонаря 1_MIR_CPY:1 ↔ Болт ГОСТ Р 50274-92 M8-6g×16-F:151
- Жесткий:337 [WeldJoint]: Крышка фонаря 1_MIR_CPY:1 ↔ Болт ГОСТ Р 50274-92 M8-6g×16-F:152
- Жесткий:338 [WeldJoint]: Крышка фонаря 1_MIR_CPY:1 ↔ Болт ГОСТ Р 50274-92 M8-6g×16-F:153
- Жесткий:339 [WeldJoint]: Крышка фонаря 1_MIR_CPY:1 ↔ Болт ГОСТ Р 50274-92 M8-6g×16-F:154
- Жесткий:340 [WeldJoint]: Крышка фонаря 1_MIR_CPY:1 ↔ Болт ГОСТ Р 50274-92 M8-6g×16-F:155
- Жесткий:341 [WeldJoint]: Крышка фонаря 1_MIR_CPY:1 ↔ Болт ГОСТ Р 50274-92 M8-6g×16-F:156
- Жесткий:342 [WeldJoint]: Крышка фонаря 1_MIR_CPY:1 ↔ Болт ГОСТ Р 50274-92 M8-6g×16-F:157
- Жесткий:343 [WeldJoint]: Крышка фонаря 1_MIR_CPY:1 ↔ Болт ГОСТ Р 50274-92 M8-6g×16-F:158
- Жесткий:344 [WeldJoint]: Крышка фонаря 1_MIR_CPY:1 ↔ Болт ГОСТ Р 50274-92 M8-6g×16-F:159
- Жесткий:345 [WeldJoint]: Крышка фонаря 1_MIR_CPY:1 ↔ Болт ГОСТ Р 50274-92 M8-6g×16-F:160
- Жесткий:346 [WeldJoint]: Крышка фонаря 1_MIR_CPY:1 ↔ Болт ГОСТ Р 50274-92 M8-6g×16-F:161
- Жесткий:347 [WeldJoint]: Крышка фонаря 1_MIR_CPY:1 ↔ Болт ГОСТ Р 50274-92 M8-6g×16-F:162
- Жесткий:348 [WeldJoint]: Крышка фонаря 1_MIR_CPY:1 ↔ Болт ГОСТ Р 50274-92 M8-6g×16-F:163
- Жесткий:349 [WeldJoint]: Крышка фонаря 1_MIR_CPY:1 ↔ Болт ГОСТ Р 50274-92 M8-6g×16-F:164
- Жесткий:350 [WeldJoint]: Крышка фонаря 1_MIR_CPY:1 ↔ Болт ГОСТ Р 50274-92 M8-6g×16-F:165
- Жесткий:351 [WeldJoint]: Крышка фонаря 1_MIR_CPY:1 ↔ Болт ГОСТ Р 50274-92 M8-6g×16-F:166
- Жесткий:352 [WeldJoint]: Крышка фонаря 2_MIR_CPY:1 ↔ Болт ГОСТ Р 50274-92 M8-6g×16-F:167
- Жесткий:353 [WeldJoint]: Крышка фонаря 2_MIR_CPY:1 ↔ Болт ГОСТ Р 50274-92 M8-6g×16-F:168
- Жесткий:354 [WeldJoint]: Крышка фонаря 2_MIR_CPY:1 ↔ Болт ГОСТ Р 50274-92 M8-6g×16-F:169
- Жесткий:355 [WeldJoint]: Крышка фонаря 2_MIR_CPY:1 ↔ Болт ГОСТ Р 50274-92 M8-6g×16-F:170
- Жесткий:356 [WeldJoint]: Крышка фонаря 2_MIR_CPY:1 ↔ Болт ГОСТ Р 50274-92 M8-6g×16-F:171
- Жесткий:357 [WeldJoint]: Крышка фонаря 2_MIR_CPY:1 ↔ Болт ГОСТ Р 50274-92 M8-6g×16-F:172
- Жесткий:358 [WeldJoint]: Крышка фонаря 2_MIR_CPY:1 ↔ Болт ГОСТ Р 50274-92 M8-6g×16-F:173
- Жесткий:359 [WeldJoint]: Крышка фонаря 2_MIR_CPY:1 ↔ Болт ГОСТ Р 50274-92 M8-6g×16-F:174
- Жесткий:360 [WeldJoint]: Крышка фонаря 2_MIR_CPY:1 ↔ Болт ГОСТ Р 50274-92 M8-6g×16-F:175
- Жесткий:361 [WeldJoint]: Крышка фонаря 2_MIR_CPY:1 ↔ Болт ГОСТ Р 50274-92 M8-6g×16-F:176
- Жесткий:362 [WeldJoint]: Крышка фонаря 1_MIR_CPY:1 ↔ Болт ГОСТ Р 50274-92 M8-6g×16-F:177
- Жесткий:363 [WeldJoint]: Крышка фонаря 1_MIR_CPY:1 ↔ Болт ГОСТ Р 50274-92 M8-6g×16-F:178
- Жесткий:364 [WeldJoint]: Крышка фонаря 2_MIR_CPY:1 ↔ Болт ГОСТ Р 50274-92 M8-6g×16-F:179
- Жесткий:365 [WeldJoint]: Крышка фонаря 2_MIR_CPY:1 ↔ Болт ГОСТ Р 50274-92 M8-6g×16-F:180
- Жесткий:366 [WeldJoint]: Крышка фонаря 2_MIR_CPY:1 ↔ Болт ГОСТ Р 50274-92 M8-6g×16-F:181
- Жесткий:367 [WeldJoint]: Крышка фонаря 1_MIR_CPY:1 ↔ Болт ГОСТ Р 50274-92 M8-6g×16-F:182
- Жесткий:368 [WeldJoint]: Крышка фонаря 2_MIR_CPY:1 ↔ Болт ГОСТ Р 50274-92 M8-6g×16-F:183
- Жесткий:369 [WeldJoint]: Крышка фонаря 2_MIR_CPY:1 ↔ Болт ГОСТ Р 50274-92 M8-6g×16-F:184
- Жесткий:370 [WeldJoint]: Крышка фонаря 2_MIR_CPY:1 ↔ Болт ГОСТ Р 50274-92 M8-6g×16-F:185
- Жесткий:371 [WeldJoint]: Крышка фонаря 2_MIR_CPY:1 ↔ Болт ГОСТ Р 50274-92 M8-6g×16-F:186
- Жесткий:372 [WeldJoint]: Крышка фонаря 2_MIR_CPY:1 ↔ Болт ГОСТ Р 50274-92 M8-6g×16-F:187
- Жесткий:373 [WeldJoint]: Крышка фонаря 2_MIR_CPY:1 ↔ Болт ГОСТ Р 50274-92 M8-6g×16-F:188
- Жесткий:374 [WeldJoint]: Крышка фонаря 2_MIR_CPY:1 ↔ Болт ГОСТ Р 50274-92 M8-6g×16-F:189
- Жесткий:375 [WeldJoint]: Крышка фонаря 2_MIR_CPY:1 ↔ Болт ГОСТ Р 50274-92 M8-6g×16-F:190
- Жесткий:376 [WeldJoint]: Крышка фонаря 2_MIR_CPY:1 ↔ Болт ГОСТ Р 50274-92 M8-6g×16-F:191
- Жесткий:377 [WeldJoint]: Крышка фонаря 2_MIR_CPY:1 ↔ Болт ГОСТ Р 50274-92 M8-6g×16-F:192